# Autodesk Inventor assembly: Bet Arm Right for 4040 - Assembly
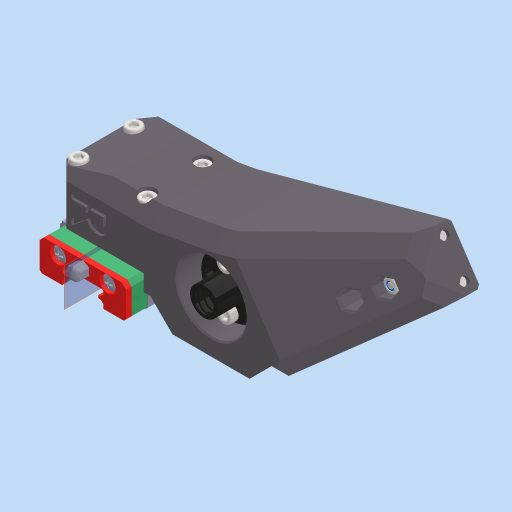
[picture p0: Inventor's stored thumbnail of the model, 512x512]
Saved by Autodesk Inventor 2023.2 (Build 272271000, 271)
## iProperties
Created: 2023-11-25
Part Number: Bet Arm Right for 4040 - Assembly
Document SubType Name: Assembly
Designer: Nils Bade
Author: Nils Bade
## Documents named in this file (12)
- C:\Users\nilsb\Documents\Inventor\Projektarbeit-Bade\RatRig_Bade\Bed Arm Right for 4040 - Assembly.iam
- C:\Users\nilsb\Documents\Inventor\Projektarbeit-Bade\RatRig_modified\Bed Arm Right for 4040.ipt
- C:\Users\nilsb\Documents\Inventor\Projektarbeit-Bade\RatRig_modified\MGN15 Linear-Rail-Block.ipt
- C:\Users\nilsb\Documents\Inventor\Projektarbeit-Bade\Schrauben\Cap Head Screw M3x20 v2.ipt
- C:\Users\nilsb\Documents\Inventor\Projektarbeit-Bade\RatRig_Standards\Magnet - 20x10x5mm - Two hole (M3 Countersink screws) v1.ipt
- C:\Users\nilsb\Documents\Inventor\Projektarbeit-Bade\Schrauben\Countersink Screw M3x12 v2.ipt
- C:\Users\nilsb\Documents\Inventor\Projektarbeit-Bade\RatRig_Standards\Hex Locking Nut - M3 v2.ipt
- C:\Users\nilsb\Documents\Inventor\Projektarbeit-Bade\RatRig_Standards\Dowel Pin - 3x35mm v1.ipt
- C:\Users\nilsb\Documents\Inventor\Projektarbeit-Bade\RatRig_Standards\Leadscrew Nut - POM - TR8_4 v1.ipt
- Leadscrew Nut - POM - TR8x8 4starts [mod].ipt
- C:\Users\nilsb\Documents\Inventor\Projektarbeit-Bade\RatRig_Standards\Rat Rig Bi-Material Lead Screw Decoupler v1.ipt
- C:\Users\nilsb\Documents\Inventor\Projektarbeit-Bade\Schrauben\Cap Head Screw M3x8 v2.ipt
## Components (19 placed, 10 different names)
1. Bed Arm Right for 4040:1 — Passend:1, Passend:2, Passend:3, Passend:4, Passend:5, Passend:6, Passend:7, Passend:8, Passend:9, Passend:10, Passend:11, Passend:12, Passend:13, Passend:14, Winkel:1, Winkel:2, Passend:21, Passend:22, Passend:23, Passend:24, Passend:25, Passend:26, Passend:27, Passend:28, Passend:29, Passend:30, Passend:31, Passend:32, Passend:35
2. MGN15 Linear-Rail-Block:1 — Passend:1, Passend:2, Passend:3
3. Cap Head Screw M3x20 v2:1 — Passend:5, Passend:11
4. Cap Head Screw M3x20 v2:2 — Passend:6, Passend:10
5. Cap Head Screw M3x20 v2:3 — Passend:7, Passend:9
6. Cap Head Screw M3x20 v2:4 — Passend:4, Passend:8
7. Magnet - 20x10x5mm - Two hole (M3 Countersink screws) v1:1 — Passend:12, Passend:13, Passend:14, Passend:15, Passend:16, Passend:17, Passend:18
8. Countersink Screw M3x12 v2:1 — Passend:15, Passend:17, Passend:20
9. Countersink Screw M3x12 v2:2 — Passend:16, Passend:18, Passend:19
10. Hex Locking Nut - M3 v2:1 — Passend:19, Winkel:1, Passend:22
11. Hex Locking Nut - M3 v2:2 — Passend:20, Winkel:2, Passend:21
12. Dowel Pin - 3x35mm v1:1 — Passend:24, Passend:25
13. Dowel Pin - 3x35mm v1:2 — Passend:23, Passend:26
14. Leadscrew Nut - POM - TR8x8 4starts [mod]:1 — Passend:30, Passend:36, Passend:37, Passend:40, Passend:41
15. Rat Rig Bi-Material Lead Screw Decoupler v1:1 — Passend:29, Passend:33, Passend:34, Passend:35, Passend:36, Passend:37, Passend:38, Passend:39
16. Cap Head Screw M3x8 v2:1 — Passend:27, Passend:32, Passend:33
17. Cap Head Screw M3x8 v2:2 — Passend:28, Passend:31, Passend:34
18. Cap Head Screw M3x8 v2:3 — Passend:38, Passend:40
19. Cap Head Screw M3x8 v2:4 — Passend:39, Passend:41
## Relationships (43: Mate 41, Angle 2)
- Passend:1 [Mate]: Bed Arm Right for 4040:1 ↔ MGN15 Linear-Rail-Block:1
- Passend:2 [Mate]: Bed Arm Right for 4040:1 ↔ MGN15 Linear-Rail-Block:1
- Passend:3 [Mate]: Bed Arm Right for 4040:1 ↔ MGN15 Linear-Rail-Block:1
- Passend:4 [Mate]: Bed Arm Right for 4040:1 ↔ Cap Head Screw M3x20 v2:4
- Passend:5 [Mate]: Bed Arm Right for 4040:1 ↔ Cap Head Screw M3x20 v2:1
- Passend:6 [Mate]: Bed Arm Right for 4040:1 ↔ Cap Head Screw M3x20 v2:2
- Passend:7 [Mate]: Bed Arm Right for 4040:1 ↔ Cap Head Screw M3x20 v2:3
- Passend:8 [Mate]: Bed Arm Right for 4040:1 ↔ Cap Head Screw M3x20 v2:4
- Passend:9 [Mate]: Bed Arm Right for 4040:1 ↔ Cap Head Screw M3x20 v2:3
- Passend:10 [Mate]: Bed Arm Right for 4040:1 ↔ Cap Head Screw M3x20 v2:2
- Passend:11 [Mate]: Bed Arm Right for 4040:1 ↔ Cap Head Screw M3x20 v2:1
- Passend:12 [Mate]: Bed Arm Right for 4040:1 ↔ Magnet - 20x10x5mm - Two hole (M3 Countersink screws) v1:1
- Passend:13 [Mate]: Bed Arm Right for 4040:1 ↔ Magnet - 20x10x5mm - Two hole (M3 Countersink screws) v1:1
- Passend:14 [Mate]: Bed Arm Right for 4040:1 ↔ Magnet - 20x10x5mm - Two hole (M3 Countersink screws) v1:1
- Passend:15 [Mate]: Magnet - 20x10x5mm - Two hole (M3 Countersink screws) v1:1 ↔ Countersink Screw M3x12 v2:1
- Passend:16 [Mate]: Magnet - 20x10x5mm - Two hole (M3 Countersink screws) v1:1 ↔ Countersink Screw M3x12 v2:2
- Passend:17 [Mate]: Magnet - 20x10x5mm - Two hole (M3 Countersink screws) v1:1 ↔ Countersink Screw M3x12 v2:1
- Passend:18 [Mate]: Magnet - 20x10x5mm - Two hole (M3 Countersink screws) v1:1 ↔ Countersink Screw M3x12 v2:2
- Passend:19 [Mate]: Countersink Screw M3x12 v2:2 ↔ Hex Locking Nut - M3 v2:1
- Passend:20 [Mate]: Countersink Screw M3x12 v2:1 ↔ Hex Locking Nut - M3 v2:2
- Winkel:1 [Angle] (0 deg): Bed Arm Right for 4040:1 ↔ Hex Locking Nut - M3 v2:1
- Winkel:2 [Angle] (0 deg): Bed Arm Right for 4040:1 ↔ Hex Locking Nut - M3 v2:2
- Passend:21 [Mate]: Bed Arm Right for 4040:1 ↔ Hex Locking Nut - M3 v2:2
- Passend:22 [Mate]: Bed Arm Right for 4040:1 ↔ Hex Locking Nut - M3 v2:1
- Passend:23 [Mate]: Bed Arm Right for 4040:1 ↔ Dowel Pin - 3x35mm v1:2
- Passend:24 [Mate]: Bed Arm Right for 4040:1 ↔ Dowel Pin - 3x35mm v1:1
- Passend:25 [Mate]: Bed Arm Right for 4040:1 ↔ Dowel Pin - 3x35mm v1:1
- Passend:26 [Mate]: Bed Arm Right for 4040:1 ↔ Dowel Pin - 3x35mm v1:2
- Passend:27 [Mate]: Bed Arm Right for 4040:1 ↔ Cap Head Screw M3x8 v2:1
- Passend:28 [Mate]: Bed Arm Right for 4040:1 ↔ Cap Head Screw M3x8 v2:2
- Passend:29 [Mate]: Bed Arm Right for 4040:1 ↔ Rat Rig Bi-Material Lead Screw Decoupler v1:1
- Passend:30 [Mate]: Bed Arm Right for 4040:1 ↔ Leadscrew Nut - POM - TR8x8 4starts [mod]:1
- Passend:31 [Mate]: Bed Arm Right for 4040:1 ↔ Cap Head Screw M3x8 v2:2
- Passend:32 [Mate]: Bed Arm Right for 4040:1 ↔ Cap Head Screw M3x8 v2:1
- Passend:33 [Mate]: Rat Rig Bi-Material Lead Screw Decoupler v1:1 ↔ Cap Head Screw M3x8 v2:1
- Passend:34 [Mate]: Rat Rig Bi-Material Lead Screw Decoupler v1:1 ↔ Cap Head Screw M3x8 v2:2
- Passend:35 [Mate]: Bed Arm Right for 4040:1 ↔ Rat Rig Bi-Material Lead Screw Decoupler v1:1
- Passend:36 [Mate]: Leadscrew Nut - POM - TR8x8 4starts [mod]:1 ↔ Rat Rig Bi-Material Lead Screw Decoupler v1:1
- Passend:37 [Mate]: Leadscrew Nut - POM - TR8x8 4starts [mod]:1 ↔ Rat Rig Bi-Material Lead Screw Decoupler v1:1
- Passend:38 [Mate]: Rat Rig Bi-Material Lead Screw Decoupler v1:1 ↔ Cap Head Screw M3x8 v2:3
- Passend:39 [Mate]: Rat Rig Bi-Material Lead Screw Decoupler v1:1 ↔ Cap Head Screw M3x8 v2:4
- Passend:40 [Mate]: Leadscrew Nut - POM - TR8x8 4starts [mod]:1 ↔ Cap Head Screw M3x8 v2:3
- Passend:41 [Mate]: Leadscrew Nut - POM - TR8x8 4starts [mod]:1 ↔ Cap Head Screw M3x8 v2:4
